# Autodesk Inventor assembly: Manipulator
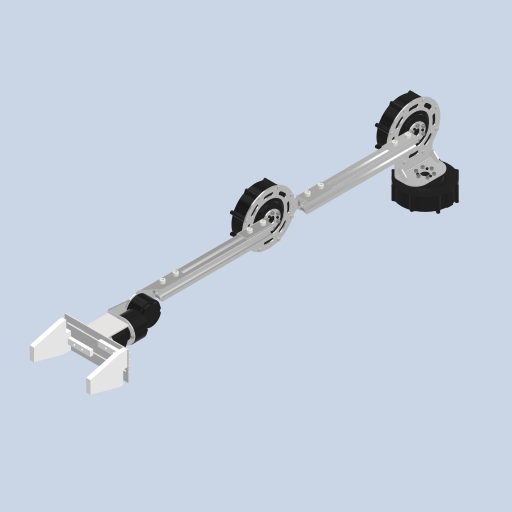
[picture p0: Inventor's stored thumbnail of the model, 512x512]
Saved by Autodesk Inventor 2023 (Build 270158000, 158)
## iProperties
Created: 2024-11-08
Part Number: Manipulator
Document SubType Name: Assembly
Designer: kiyo
Author: kiyo
## Documents named in this file (18)
- D:\GitHub\inventor\syu-si\OfficeRobot\Manipulator\Manipulator.iam
- D:\GitHub\inventor\syu-si\OfficeRobot\ReadyMade\Steadywin\GIM8108-8.iam
- D:\GitHub\inventor\syu-si\OfficeRobot\Manipulator\elbow-pitch-bracket.ipt
- D:\GitHub\inventor\syu-si\OfficeRobot\ReadyMade\Screw\M3_6mm.ipt
- D:\GitHub\inventor\syu-si\OfficeRobot\ReadyMade\Steadywin\GIM3505-8_with-driver.ipt
- D:\GitHub\inventor\syu-si\OfficeRobot\Manipulator\wrist_roll_plate.ipt
- D:\GitHub\inventor\syu-si\OfficeRobot\Manipulator\wrist-pitch-plate.ipt
- D:\GitHub\inventor\syu-si\OfficeRobot\ReadyMade\Screw\M2-5_6mm.ipt
- D:\GitHub\inventor\syu-si\OfficeRobot\ReadyMade\Screw\CBSH3-8.ipt
- D:\GitHub\inventor\syu-si\OfficeRobot\ReadyMade\Screw\FWSJJ-D5-V2_6-T4_5.ipt
- D:\GitHub\inventor\syu-si\OfficeRobot\ReadyMade\Screw\M2-5_10mm.ipt
- D:\GitHub\inventor\syu-si\OfficeRobot\ReadyMade\Screw\HNTU5-5.ipt
- D:\GitHub\inventor\syu-si\OfficeRobot\Manipulator\pitch_plate_20mm.ipt
- D:\GitHub\inventor\syu-si\OfficeRobot\ReadyMade\Aluminum-frame\HFS5-2020-210-AV10-BV35-CV175-DV200.ipt
- D:\GitHub\inventor\syu-si\OfficeRobot\Manipulator\sholder_roll_bracket.ipt
- D:\GitHub\inventor\syu-si\OfficeRobot\ReadyMade\Screw\SCB5-22.ipt
- D:\GitHub\inventor\syu-si\OfficeRobot\ReadyMade\Screw\SCB5-8.ipt
- D:\GitHub\inventor\syu-si\OfficeRobot\Manipulator\Hand_tyokudou.iam
## Components (87 placed, 17 different names)
1. pitch_plate_20mm:1 — フラッシュ:1, 挿入:355, 挿入:356, 挿入:357, 挿入:358, 挿入:359, 挿入:360, 角度:47
2. pitch_plate_20mm:2 — 挿入:345, フラッシュ:3, 角度:40
3. elbow-pitch-bracket:1 — 挿入:341, 挿入:342, フラッシュ:2, フラッシュ:7, フラッシュ:8
4. sholder_roll_bracket:1 — 挿入:350, 挿入:361, 挿入:362, 挿入:363, 挿入:364, 挿入:365, 挿入:366, 挿入:414, 挿入:415
5. HFS5-2020-210-AV10-BV35-CV175-DV200:1 — フラッシュ:1, フラッシュ:2, メイト:19, メイト:20, 角度:35, 角度:36, メイト:21, メイト:22, フラッシュ:9, 角度:37, メイト:23, メイト:24
6. HFS5-2020-210-AV10-BV35-CV175-DV200:2 — フラッシュ:3, 挿入:351, 挿入:352, 角度:27, 角度:28, 挿入:353, 挿入:354, 角度:29, 角度:30, メイト:15, メイト:16, 角度:33, フラッシュ:5, メイト:17, メイト:18, 角度:34, フラッシュ:6, メイト:25, メイト:26, メイト:27, メイト:28, メイト:29, メイト:30
7. wrist-pitch-plate:1 — 挿入:409, 挿入:410, メイト:29, メイト:30, 正接:1, 正接:2, 正接:3
8. wrist_roll_plate:2 — 挿入:402, 挿入:403, 挿入:404, 挿入:405, 挿入:406, 挿入:407, 挿入:408, 挿入:413
9. Hand_tyokudou:1 [sub-assembly] — 挿入:413, 角度:45
10. M3_6mm:7 — 挿入:337
11. M3_6mm:8 — 挿入:336
12. M3_6mm:9 — 挿入:334
13. M3_6mm:10 — 挿入:338
14. M3_6mm:11 — 挿入:339
15. M3_6mm:12 — 挿入:335
16. M3_6mm:19 — 挿入:358
17. M3_6mm:20 — 挿入:357
18. M3_6mm:21 — 挿入:355
19. M3_6mm:22 — 挿入:356
20. M3_6mm:23 — 挿入:359
21. M3_6mm:24 — 挿入:360
22. M3_6mm:25 — 挿入:361
23. M3_6mm:26 — 挿入:363
24. M3_6mm:27 — 挿入:362
25. M3_6mm:28 — 挿入:364
26. M3_6mm:29 — 挿入:365
27. M3_6mm:30 — 挿入:366
28. CBSH3-8:1 — 挿入:307
29. CBSH3-8:2 — 挿入:308
30. CBSH3-8:3 — 挿入:302
31. CBSH3-8:4 — 挿入:304, 挿入:415
32. CBSH3-8:5 — 挿入:309
33. CBSH3-8:6 — 挿入:303
34. CBSH3-8:7 — 挿入:305
35. CBSH3-8:8 — 挿入:306
36. CBSH3-8:9 — 挿入:332
37. CBSH3-8:10 — 挿入:327
38. CBSH3-8:11 — 挿入:330
39. CBSH3-8:12 — 挿入:328
40. CBSH3-8:13 — 挿入:329
41. CBSH3-8:14 — 挿入:331
42. CBSH3-8:15 — 挿入:326
43. CBSH3-8:16 — 挿入:333
44. M2-5_6mm:13
45. M2-5_6mm:14
46. M2-5_6mm:15
47. M2-5_10mm:7 — 挿入:402
48. M2-5_10mm:8 — 挿入:403
49. M2-5_10mm:9 — 挿入:404
50. FWSJJ-D5-V2_6-T4_5:10 — 挿入:407
51. FWSJJ-D5-V2_6-T4_5:11 — 挿入:405
52. FWSJJ-D5-V2_6-T4_5:12 — 挿入:406
53. HNTU5-5:22 — 挿入:412, メイト:27, メイト:28
54. SCB5-8:8 — 挿入:412, 正接:2
55. HNTU5-5:23 — 挿入:411, メイト:25, メイト:26
56. SCB5-8:9 — 挿入:411, 正接:3
57. SCB5-22:1 — 挿入:368
58. SCB5-22:2 — 挿入:367
59. SCB5-22:3 — 挿入:370
60. SCB5-22:4 — 挿入:369
61. SCB5-22:5 — 挿入:372
62. SCB5-22:6 — 挿入:371
63. SCB5-22:7 — 挿入:376
64. SCB5-22:8 — 挿入:375, 正接:1
65. SCB5-8:3
66. SCB5-8:4
67. SCB5-8:5
68. SCB5-8:6
69. SCB5-8:7
70. HNTU5-5:6 — 挿入:372
71. HNTU5-5:7 — 挿入:371
72. HNTU5-5:9 — 挿入:369
73. HNTU5-5:10 — 挿入:370
74. HNTU5-5:11 — 挿入:351, 角度:28, 挿入:367
75. HNTU5-5:12 — 挿入:352, 角度:27, 挿入:368
76. HNTU5-5:13 — 挿入:353, 角度:30, 挿入:376
77. HNTU5-5:14 — 挿入:354, 角度:29, 挿入:375
78. HNTU5-5:17 — メイト:15, メイト:16, 角度:33, フラッシュ:5
79. HNTU5-5:18 — メイト:17, メイト:18, 角度:34, フラッシュ:6
80. HNTU5-5:19 — フラッシュ:8, メイト:19, メイト:20, 角度:35
81. HNTU5-5:20 — フラッシュ:7, 角度:36, メイト:21, メイト:22
82. HNTU5-5:21 — フラッシュ:9, 角度:37, メイト:23, メイト:24
83. GIM8108-8:1 [sub-assembly] — 挿入:350, 角度:46, 角度:48
84. GIM8108-8:2 [sub-assembly] — 挿入:302, 挿入:303, 挿入:304, 挿入:305, 挿入:306, 挿入:307, 挿入:308, 挿入:309, 角度:46, 挿入:414, 角度:47
85. GIM8108-8:3 [sub-assembly] — 挿入:326, 挿入:327, 挿入:328, 挿入:329, 挿入:330, 挿入:331, 挿入:332, 挿入:333, 挿入:334, 挿入:335, 挿入:336, 挿入:337, 挿入:338, 挿入:339, 挿入:341, 挿入:342, 挿入:345, 角度:40
86. GIM3505-8_with-driver:9 — 挿入:408, 挿入:409, 挿入:410, 角度:44
87. GIM3505-8_with-driver:8 — 角度:44, 角度:45
## Relationships (132: Insert 79, Mate 22, Angle 20, Flush 8, Tangent 3)
- 挿入:302 [Insert] (2 mm): CBSH3-8:3 ↔ GIM8108-8:2
- 挿入:303 [Insert] (2 mm): CBSH3-8:6 ↔ GIM8108-8:2
- 挿入:304 [Insert] (2 mm): CBSH3-8:4 ↔ GIM8108-8:2
- 挿入:305 [Insert] (2 mm): CBSH3-8:7 ↔ GIM8108-8:2
- 挿入:306 [Insert] (2 mm): CBSH3-8:8 ↔ GIM8108-8:2
- 挿入:307 [Insert] (2 mm): CBSH3-8:1 ↔ GIM8108-8:2
- 挿入:308 [Insert] (2 mm): CBSH3-8:2 ↔ GIM8108-8:2
- 挿入:309 [Insert] (2 mm): CBSH3-8:5 ↔ GIM8108-8:2
- [Insert] (-0.75 mm): HFS5-2020-210-AV10-BV35-CV175-DV200:1 ↔ HNTU5-5:6
- [Angle] (0 deg): HFS5-2020-210-AV10-BV35-CV175-DV200:1 ↔ HNTU5-5:6
- [Insert] (-0.75 mm): HFS5-2020-210-AV10-BV35-CV175-DV200:1 ↔ HNTU5-5:7
- [Angle] (0 deg): HFS5-2020-210-AV10-BV35-CV175-DV200:1 ↔ HNTU5-5:7
- [Angle] (0 deg): HFS5-2020-210-AV10-BV35-CV175-DV200:1 ↔ HNTU5-5:6
- 挿入:326 [Insert] (2 mm): CBSH3-8:15 ↔ GIM8108-8:3
- 挿入:327 [Insert] (2 mm): CBSH3-8:10 ↔ GIM8108-8:3
- 挿入:328 [Insert] (2 mm): CBSH3-8:12 ↔ GIM8108-8:3
- 挿入:329 [Insert] (2 mm): CBSH3-8:13 ↔ GIM8108-8:3
- 挿入:330 [Insert] (2 mm): CBSH3-8:11 ↔ GIM8108-8:3
- 挿入:331 [Insert] (2 mm): CBSH3-8:14 ↔ GIM8108-8:3
- 挿入:332 [Insert] (2 mm): CBSH3-8:9 ↔ GIM8108-8:3
- 挿入:333 [Insert] (2 mm): CBSH3-8:16 ↔ GIM8108-8:3
- 挿入:334 [Insert] (2 mm): M3_6mm:9 ↔ GIM8108-8:3
- 挿入:335 [Insert] (2 mm): M3_6mm:12 ↔ GIM8108-8:3
- 挿入:336 [Insert] (2 mm): M3_6mm:8 ↔ GIM8108-8:3
- 挿入:337 [Insert] (2 mm): M3_6mm:7 ↔ GIM8108-8:3
- 挿入:338 [Insert] (2 mm): M3_6mm:10 ↔ GIM8108-8:3
- 挿入:339 [Insert] (2 mm): M3_6mm:11 ↔ GIM8108-8:3
- [Insert]: pitch_plate_20mm:1 ↔ GIM8108-8:2
- [Mate]: pitch_plate_20mm:1 ↔ HFS5-2020-210-AV10-BV35-CV175-DV200:1
- [Mate]: pitch_plate_20mm:1 ↔ HFS5-2020-210-AV10-BV35-CV175-DV200:1
- 挿入:341 [Insert]: elbow-pitch-bracket:1 ↔ GIM8108-8:3
- 挿入:342 [Insert]: elbow-pitch-bracket:1 ↔ GIM8108-8:3
- [Angle] (0 deg): HFS5-2020-210-AV10-BV35-CV175-DV200:1 ↔ HNTU5-5:9
- [Angle] (0 deg): HFS5-2020-210-AV10-BV35-CV175-DV200:1 ↔ HNTU5-5:10
- [Insert] (-0.75 mm): HFS5-2020-210-AV10-BV35-CV175-DV200:1 ↔ HNTU5-5:9
- [Insert] (-0.75 mm): HFS5-2020-210-AV10-BV35-CV175-DV200:1 ↔ HNTU5-5:10
- [Mate]: elbow-pitch-bracket:1 ↔ HFS5-2020-210-AV10-BV35-CV175-DV200:1
- [Mate]: elbow-pitch-bracket:1 ↔ HFS5-2020-210-AV10-BV35-CV175-DV200:1
- 挿入:345 [Insert]: pitch_plate_20mm:2 ↔ GIM8108-8:3
- [Mate]: pitch_plate_20mm:2 ↔ HFS5-2020-210-AV10-BV35-CV175-DV200:2
- [Mate]: pitch_plate_20mm:2 ↔ HFS5-2020-210-AV10-BV35-CV175-DV200:2
- 挿入:350 [Insert]: sholder_roll_bracket:1 ↔ GIM8108-8:1
- フラッシュ:1 [Flush]: pitch_plate_20mm:1 ↔ HFS5-2020-210-AV10-BV35-CV175-DV200:1
- フラッシュ:2 [Flush]: elbow-pitch-bracket:1 ↔ HFS5-2020-210-AV10-BV35-CV175-DV200:1
- フラッシュ:3 [Flush]: pitch_plate_20mm:2 ↔ HFS5-2020-210-AV10-BV35-CV175-DV200:2
- 挿入:351 [Insert] (-0.75 mm): HFS5-2020-210-AV10-BV35-CV175-DV200:2 ↔ HNTU5-5:11
- 挿入:352 [Insert] (-0.75 mm): HFS5-2020-210-AV10-BV35-CV175-DV200:2 ↔ HNTU5-5:12
- 角度:27 [Angle] (0 deg): HFS5-2020-210-AV10-BV35-CV175-DV200:2 ↔ HNTU5-5:12
- 角度:28 [Angle] (0 deg): HFS5-2020-210-AV10-BV35-CV175-DV200:2 ↔ HNTU5-5:11
- 挿入:353 [Insert] (-0.75 mm): HFS5-2020-210-AV10-BV35-CV175-DV200:2 ↔ HNTU5-5:13
- 挿入:354 [Insert] (-0.75 mm): HFS5-2020-210-AV10-BV35-CV175-DV200:2 ↔ HNTU5-5:14
- 角度:29 [Angle] (0 deg): HFS5-2020-210-AV10-BV35-CV175-DV200:2 ↔ HNTU5-5:14
- 角度:30 [Angle] (0 deg): HFS5-2020-210-AV10-BV35-CV175-DV200:2 ↔ HNTU5-5:13
- 挿入:355 [Insert]: pitch_plate_20mm:1 ↔ M3_6mm:21
- 挿入:356 [Insert]: pitch_plate_20mm:1 ↔ M3_6mm:22
- 挿入:357 [Insert]: pitch_plate_20mm:1 ↔ M3_6mm:20
- 挿入:358 [Insert]: pitch_plate_20mm:1 ↔ M3_6mm:19
- 挿入:359 [Insert]: pitch_plate_20mm:1 ↔ M3_6mm:23
- 挿入:360 [Insert]: pitch_plate_20mm:1 ↔ M3_6mm:24
- 挿入:361 [Insert]: sholder_roll_bracket:1 ↔ M3_6mm:25
- 挿入:362 [Insert]: sholder_roll_bracket:1 ↔ M3_6mm:27
- 挿入:363 [Insert]: sholder_roll_bracket:1 ↔ M3_6mm:26
- 挿入:364 [Insert]: sholder_roll_bracket:1 ↔ M3_6mm:28
- 挿入:365 [Insert]: sholder_roll_bracket:1 ↔ M3_6mm:29
- 挿入:366 [Insert]: sholder_roll_bracket:1 ↔ M3_6mm:30
- 挿入:367 [Insert] (-1.25 mm): SCB5-22:2 ↔ HNTU5-5:11
- 挿入:368 [Insert] (-1.25 mm): SCB5-22:1 ↔ HNTU5-5:12
- 挿入:369 [Insert] (-1.25 mm): SCB5-22:4 ↔ HNTU5-5:9
- 挿入:370 [Insert] (-1.25 mm): SCB5-22:3 ↔ HNTU5-5:10
- 挿入:371 [Insert] (-1.25 mm): SCB5-22:6 ↔ HNTU5-5:7
- 挿入:372 [Insert] (-1.25 mm): SCB5-22:5 ↔ HNTU5-5:6
- 挿入:375 [Insert] (-1.25 mm): SCB5-22:8 ↔ HNTU5-5:14
- 挿入:376 [Insert] (-1.25 mm): SCB5-22:7 ↔ HNTU5-5:13
- [Insert] (3.2 mm): SCB5-8:3 ↔ HNTU5-5:17
- メイト:15 [Mate]: HFS5-2020-210-AV10-BV35-CV175-DV200:2 ↔ HNTU5-5:17
- メイト:16 [Mate] (1 mm): HFS5-2020-210-AV10-BV35-CV175-DV200:2 ↔ HNTU5-5:17
- 角度:33 [Angle] (0 deg): HFS5-2020-210-AV10-BV35-CV175-DV200:2 ↔ HNTU5-5:17
- フラッシュ:5 [Flush] (33.5 mm): HFS5-2020-210-AV10-BV35-CV175-DV200:2 ↔ HNTU5-5:17
- [Insert] (3.2 mm): SCB5-8:4 ↔ HNTU5-5:18
- メイト:17 [Mate]: HFS5-2020-210-AV10-BV35-CV175-DV200:2 ↔ HNTU5-5:18
- メイト:18 [Mate] (1 mm): HFS5-2020-210-AV10-BV35-CV175-DV200:2 ↔ HNTU5-5:18
- 角度:34 [Angle] (0 deg): HFS5-2020-210-AV10-BV35-CV175-DV200:2 ↔ HNTU5-5:18
- フラッシュ:6 [Flush] (33.5 mm): HFS5-2020-210-AV10-BV35-CV175-DV200:2 ↔ HNTU5-5:18
- [Insert] (3.2 mm): SCB5-8:5 ↔ HNTU5-5:19
- [Insert] (3.2 mm): SCB5-8:6 ↔ HNTU5-5:20
- フラッシュ:7 [Flush] (5.5 mm): elbow-pitch-bracket:1 ↔ HNTU5-5:20
- フラッシュ:8 [Flush] (-30.5 mm): elbow-pitch-bracket:1 ↔ HNTU5-5:19
- メイト:19 [Mate]: HFS5-2020-210-AV10-BV35-CV175-DV200:1 ↔ HNTU5-5:19
- メイト:20 [Mate] (1 mm): HFS5-2020-210-AV10-BV35-CV175-DV200:1 ↔ HNTU5-5:19
- 角度:35 [Angle] (0 deg): HFS5-2020-210-AV10-BV35-CV175-DV200:1 ↔ HNTU5-5:19
- 角度:36 [Angle] (0 deg): HFS5-2020-210-AV10-BV35-CV175-DV200:1 ↔ HNTU5-5:20
- メイト:21 [Mate] (1 mm): HFS5-2020-210-AV10-BV35-CV175-DV200:1 ↔ HNTU5-5:20
- メイト:22 [Mate]: HFS5-2020-210-AV10-BV35-CV175-DV200:1 ↔ HNTU5-5:20
- [Insert] (3.2 mm): SCB5-8:7 ↔ HNTU5-5:21
- フラッシュ:9 [Flush] (33.5 mm): HFS5-2020-210-AV10-BV35-CV175-DV200:1 ↔ HNTU5-5:21
- 角度:37 [Angle] (0 deg): HFS5-2020-210-AV10-BV35-CV175-DV200:1 ↔ HNTU5-5:21
- メイト:23 [Mate] (1 mm): HFS5-2020-210-AV10-BV35-CV175-DV200:1 ↔ HNTU5-5:21
- メイト:24 [Mate]: HFS5-2020-210-AV10-BV35-CV175-DV200:1 ↔ HNTU5-5:21
- 角度:40 [Angle] (0 deg): pitch_plate_20mm:2 ↔ GIM8108-8:3
- [Insert]: wrist_roll_plate:2 ↔ M2-5_6mm:13
- [Insert]: wrist_roll_plate:2 ↔ M2-5_6mm:14
- [Insert]: wrist_roll_plate:2 ↔ M2-5_6mm:15
- [Insert]: wrist_roll_plate:2 ↔ GIM3505-8_with-driver:8
- [Insert]: wrist_roll_plate:2 ↔ GIM3505-8_with-driver:8
- 挿入:402 [Insert]: wrist_roll_plate:2 ↔ M2-5_10mm:7
- 挿入:403 [Insert]: wrist_roll_plate:2 ↔ M2-5_10mm:8
- 挿入:404 [Insert]: wrist_roll_plate:2 ↔ M2-5_10mm:9
- 挿入:405 [Insert]: wrist_roll_plate:2 ↔ FWSJJ-D5-V2_6-T4_5:11
- 挿入:406 [Insert]: wrist_roll_plate:2 ↔ FWSJJ-D5-V2_6-T4_5:12
- 挿入:407 [Insert]: wrist_roll_plate:2 ↔ FWSJJ-D5-V2_6-T4_5:10
- 挿入:408 [Insert] (3.5 mm): wrist_roll_plate:2 ↔ GIM3505-8_with-driver:9
- 挿入:409 [Insert]: wrist-pitch-plate:1 ↔ GIM3505-8_with-driver:9
- 挿入:410 [Insert]: wrist-pitch-plate:1 ↔ GIM3505-8_with-driver:9
- 挿入:411 [Insert] (3.2 mm): HNTU5-5:23 ↔ SCB5-8:9
- 挿入:412 [Insert] (3.2 mm): HNTU5-5:22 ↔ SCB5-8:8
- メイト:25 [Mate]: HFS5-2020-210-AV10-BV35-CV175-DV200:2 ↔ HNTU5-5:23
- メイト:26 [Mate] (1 mm): HFS5-2020-210-AV10-BV35-CV175-DV200:2 ↔ HNTU5-5:23
- メイト:27 [Mate] (1 mm): HFS5-2020-210-AV10-BV35-CV175-DV200:2 ↔ HNTU5-5:22
- メイト:28 [Mate]: HFS5-2020-210-AV10-BV35-CV175-DV200:2 ↔ HNTU5-5:22
- メイト:29 [Mate]: HFS5-2020-210-AV10-BV35-CV175-DV200:2 ↔ wrist-pitch-plate:1
- メイト:30 [Mate]: HFS5-2020-210-AV10-BV35-CV175-DV200:2 ↔ wrist-pitch-plate:1
- 正接:1 [Tangent] (0.25 mm): wrist-pitch-plate:1 ↔ SCB5-22:8
- 正接:2 [Tangent] (0.25 mm): wrist-pitch-plate:1 ↔ SCB5-8:8
- 正接:3 [Tangent] (0.25 mm): wrist-pitch-plate:1 ↔ SCB5-8:9
- 挿入:413 [Insert] (10 mm): wrist_roll_plate:2 ↔ Hand_tyokudou:1
- 角度:44 [Angle] (0 deg): GIM3505-8_with-driver:9 ↔ GIM3505-8_with-driver:8
- 角度:45 [Angle] (0 deg): Hand_tyokudou:1 ↔ GIM3505-8_with-driver:8
- 角度:46 [Angle] (0 deg): GIM8108-8:1 ↔ GIM8108-8:2
- 挿入:414 [Insert]: sholder_roll_bracket:1 ↔ GIM8108-8:2
- 挿入:415 [Insert]: sholder_roll_bracket:1 ↔ CBSH3-8:4
- 角度:47 [Angle] (0 deg): pitch_plate_20mm:1 ↔ GIM8108-8:2
- 角度:48 [Angle] (0 deg): GIM8108-8:1
## Named parameters: d472_d466 = 3.2 mm, d477_d466 = 3.2 mm, d482_d466 = 3.2 mm, d483_d466 = 3.2 mm, d492_d466 = 3.2 mm, d516_d512 = 0 mm, d517_d513 = 0 mm, d519_d268 = 0 mm, d520_d269 = 0 mm, d521_d270 = 0 mm
